# Autodesk Inventor assembly: battery
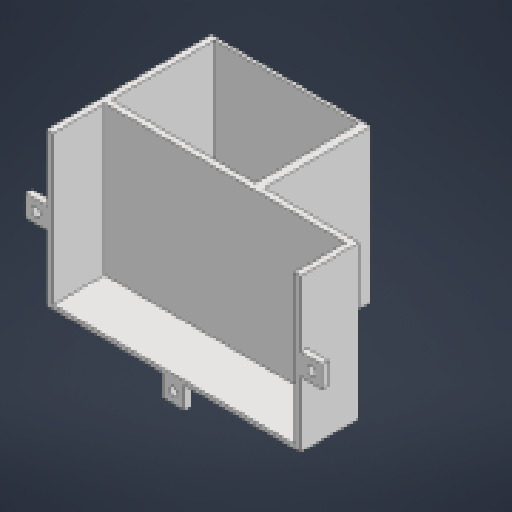
[picture p0: Inventor's stored thumbnail of the model, 512x512]
Saved by Autodesk Inventor 2026.1 (Build 301233020, 233B)
## iProperties
Created: 2025-11-26
Part Number: battery
Document SubType Name: Assembly
Designer: jaewook
Author: jaewook
## Documents named in this file (4)
- C:\Users\kjh19\Documents\Inventor\project\final\base_device\battery.iam
- C:\Users\kjh19\Documents\Inventor\project\final\base_device\battery_1.ipt
- C:\Users\kjh19\Documents\Inventor\project\final\base_device\battery_2.ipt
- C:\Users\kjh19\Documents\Inventor\project\final\battery_base.ipt
## Components (3 placed, 3 different names)
1. battery_1:1 — 강체:1
2. battery_2:1 — 강체:2
3. battery_base:1 — 강체:1, 강체:2
## Relationships (2: WeldJoint 2)
- 강체:1 [WeldJoint]: battery_1:1 ↔ battery_base:1
- 강체:2 [WeldJoint]: battery_2:1 ↔ battery_base:1
